# Autodesk Inventor assembly: Z assembly
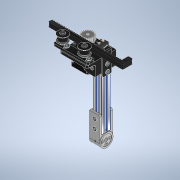
[picture p0: Inventor's stored thumbnail of the model, 180x180]
Saved by Autodesk Inventor 2022 (Build 260153000, 153)
## iProperties
Created: 2022-03-06
Part Number: Z assembly
Document SubType Name: Assembly
Designer: JK
Author: JK
## Documents named in this file (26)
- C:\Users\JK\Documents\Inventor\ScaraNema\SCARA-3DP\Parts\Forearm\Forearm assembly.iam
- C:\Users\JK\Documents\Inventor\ScaraNema\SCARA-3DP\Parts\Forearm\Z Motor support.ipt
- C:\Users\JK\Documents\Inventor\ScaraNema\SCARA-3DP\Parts\Forearm\Gear.ipt
- C:\Users\JK\Documents\Inventor\ScaraNema\SCARA-3DP\Parts\Forearm\Rack.ipt
- C:\Users\JK\Documents\Inventor\ScaraNema\SCARA-3DP\Parts\Common components\Motor.ipt
- C:\Users\JK\Documents\Inventor\ScaraNema\SCARA-3DP\Parts\V-Slot 20x20.ipt
- C:\Users\JK\Documents\Inventor\ScaraNema\SCARA-3DP\Parts\Forearm\Rack support.ipt
- C:\Users\JK\Documents\Inventor\ScaraNema\SCARA-3DP\Parts\Forearm\Roller.ipt
- C:\Users\JK\Documents\Inventor\ScaraNema\SCARA-3DP\Parts\Forearm\Z axis limit switch support.ipt
- C:\Users\JK\Documents\Inventor\ScaraNema\SCARA-3DP\Parts\Common components\V-Slot 20x20\V-Slot 20x20x150.ipt
- C:\Users\JK\Documents\Inventor\ScaraNema\SCARA-3DP\Parts\Arm\Soporte antebrazo.ipt
- C:\Users\JK\Documents\Inventor\ScaraNema\SCARA-3DP\Parts\Common components\Limit switch.ipt
- C:\Users\JK\Documents\Inventor\ScaraNema\SCARA-3DP\Parts\Fasteners\M2x10 socket bolt.ipt
- C:\Users\JK\Documents\Inventor\ScaraNema\SCARA-3DP\Parts\Fasteners\M2 Hex nut.ipt
- C:\Users\JK\Documents\Inventor\ScaraNema\SCARA-3DP\Parts\Fasteners\M3x10 set screw.ipt
- C:\Users\JK\Documents\Inventor\ScaraNema\SCARA-3DP\Parts\Fasteners\M5x15 Flat head bolt.ipt
- C:\Users\JK\Documents\Inventor\ScaraNema\SCARA-3DP\Parts\Fasteners\M5x10 Flat head bolt.ipt
- C:\Users\JK\Documents\Inventor\ScaraNema\SCARA-3DP\Parts\Fasteners\M5x8 Flat head bolt.ipt
- C:\Users\JK\Documents\Inventor\ScaraNema\SCARA-3DP\Parts\Fasteners\M3 Hex nut.ipt
- C:\Users\JK\Documents\Inventor\ScaraNema\SCARA-3DP\Parts\Fasteners\M5 Hex nut.ipt
- C:\Users\JK\Documents\Inventor\ScaraNema\SCARA-3DP\Parts\Common components\688-2RS.ipt
- C:\Users\JK\Documents\Inventor\ScaraNema\SCARA-3DP\Parts\Forearm\F623ZZ.ipt
- C:\Users\JK\Documents\Inventor\ScaraNema\SCARA-3DP\Parts\Fasteners\M3x25 socket solt.ipt
- C:\Users\JK\Documents\Inventor\ScaraNema\SCARA-3DP\Parts\Fasteners\M5 T-Nut Drop-in 20x20.ipt
- C:\Users\JK\Documents\Inventor\ScaraNema\SCARA-3DP\Parts\Forearm\Roller-bolt separator.ipt
- C:\Users\JK\Documents\Inventor\ScaraNema\SCARA-3DP\Parts\Fasteners\M3x6 socket bolt.ipt
## Components (61 placed, 24 different names)
1. Z Motor support:1 — Ángulo:2, Coincidencia:3, Ángulo:3, Coincidencia:4, Coincidencia:5, Nivelación:1, Coincidencia:6, Coincidencia:7, Nivelación:5, Coincidencia:32, Coincidencia:48, Coincidencia:49, Coincidencia:50, Coincidencia:51, Coincidencia:52, Ángulo:9, Coincidencia:56, Ángulo:19, Coincidencia:91, Coincidencia:92, Coincidencia:93, Coincidencia:94, Coincidencia:95, Coincidencia:96
2. Gear:1 — Coincidencia:1, Coincidencia:2, Coincidencia:3, Nivelación:2
3. Rack:1 — Ángulo:2, Nivelación:2, Nivelación:3, Tangente:1
4. Motor:1 — Coincidencia:1, Coincidencia:2, Ángulo:3, Coincidencia:4, Nivelación:3
5. V-Slot 20x20x150:1 — Coincidencia:5, Nivelación:1, Coincidencia:6, Coincidencia:16, Nivelación:8, Coincidencia:17, Coincidencia:18, Coincidencia:19, Coincidencia:29, Ángulo:12
6. Rack support:1 — Coincidencia:7, Nivelación:5, Coincidencia:39, Coincidencia:40, Ángulo:6, Coincidencia:41, Coincidencia:53, Coincidencia:61, Coincidencia:62, Coincidencia:63
7. Roller:1 — Nivelación:7, Tangente:1, Coincidencia:57, Coincidencia:60, Coincidencia:61, Nivelación:18, Coincidencia:64, Coincidencia:66
8. Roller:2 — Nivelación:7, Coincidencia:58, Coincidencia:59, Coincidencia:62, Nivelación:18, Coincidencia:65
9. Z axis limit switch support:1 — Coincidencia:16, Nivelación:8, Coincidencia:20, Coincidencia:21, Coincidencia:22, Ángulo:5, Coincidencia:28, Coincidencia:29, Coincidencia:46, Coincidencia:47, Coincidencia:89, Coincidencia:90
10. Soporte antebrazo:1 — Coincidencia:17, Coincidencia:18, Coincidencia:19, Coincidencia:33, Coincidencia:34, Coincidencia:35, Coincidencia:36, Coincidencia:37, Coincidencia:38, Coincidencia:42, Ángulo:8, Coincidencia:43, Coincidencia:44, Coincidencia:45, Ángulo:15, Coincidencia:83, Coincidencia:84, Coincidencia:85, Coincidencia:86, Coincidencia:87, Coincidencia:88
11. Limit switch:1 — Coincidencia:20, Coincidencia:21, Coincidencia:22, Coincidencia:23, Coincidencia:24, Coincidencia:25
12. M2x10 socket bolt:1 — Coincidencia:23, Nivelación:9, Coincidencia:26
13. M2x10 socket bolt:2 — Coincidencia:24, Nivelación:9, Coincidencia:25, Coincidencia:27
14. M2 Hex nut:1 — Coincidencia:27, Nivelación:10, Ángulo:4, Ángulo:5
15. M2 Hex nut:2 — Coincidencia:26, Nivelación:10, Ángulo:4, Coincidencia:28
16. M5x15 Flat head bolt:1 — Coincidencia:32, Coincidencia:73, Coincidencia:93
17. M5x10 Flat head bolt:1 — Coincidencia:33, Nivelación:12, Coincidencia:82, Coincidencia:86
18. M5x10 Flat head bolt:2 — Coincidencia:34, Nivelación:12, Coincidencia:81
19. M5x10 Flat head bolt:3 — Coincidencia:35, Nivelación:11, Coincidencia:77, Coincidencia:88
20. M5x10 Flat head bolt:4 — Coincidencia:36, Nivelación:11, Coincidencia:78
21. M5x8 Flat head bolt:1 — Coincidencia:37, Nivelación:13, Coincidencia:79, Coincidencia:87
22. M5x8 Flat head bolt:2 — Coincidencia:38, Nivelación:13, Coincidencia:80
23. M3 Hex nut:2 — Coincidencia:40, Nivelación:14, Ángulo:6, Ángulo:7, Coincidencia:41
24. M3 Hex nut:3 — Coincidencia:39, Nivelación:14, Ángulo:7
25. M5x8 Flat head bolt:3 — Coincidencia:47, Nivelación:15, Coincidencia:75, Coincidencia:90
26. M5x8 Flat head bolt:4 — Coincidencia:46, Nivelación:15, Coincidencia:74
27. M5x15 Flat head bolt:2 — Coincidencia:48, Coincidencia:76, Coincidencia:94
28. M5x15 Flat head bolt:3 — Coincidencia:49, Coincidencia:50
29. M5x10 Flat head bolt:5 — Coincidencia:52, Nivelación:16, Coincidencia:54
30. M5x10 Flat head bolt:6 — Coincidencia:51, Nivelación:16, Coincidencia:53, Coincidencia:55
31. M5 Hex nut:1 — Coincidencia:54, Nivelación:17, Ángulo:9, Ángulo:10
32. M5 Hex nut:2 — Coincidencia:55, Nivelación:17, Ángulo:10, Coincidencia:56
33. 688-2RS:1 — Coincidencia:57, Coincidencia:60, Coincidencia:63
34. 688-2RS:2 — Coincidencia:58, Coincidencia:59
35. F623ZZ:1 — Coincidencia:64, Nivelación:19, Coincidencia:66, Coincidencia:67, Coincidencia:69, Coincidencia:70
36. F623ZZ:2 — Coincidencia:65, Nivelación:19, Coincidencia:68
37. Roller-bolt separator:1 — Coincidencia:67, Coincidencia:69, Nivelación:20, Coincidencia:72
38. Roller-bolt separator:2 — Coincidencia:68, Nivelación:20, Coincidencia:71
39. M3x25 socket solt:1 — Coincidencia:71, Nivelación:21
40. M3x25 socket solt:2 — Coincidencia:70, Nivelación:21, Coincidencia:72
41. M5 T-Nut Drop-in 20x20:1 — Coincidencia:73, Coincidencia:91
42. M5 T-Nut Drop-in 20x20:2 — Coincidencia:74, Nivelación:22, Ángulo:18, Ángulo:19
43. M5 T-Nut Drop-in 20x20:3 — Coincidencia:75, Nivelación:22, Ángulo:18, Coincidencia:89
44. M5 T-Nut Drop-in 20x20:4 — Coincidencia:76, Coincidencia:92
45. M5 T-Nut Drop-in 20x20:5 — Coincidencia:77, Ángulo:13, Nivelación:25, Ángulo:14, Ángulo:17, Coincidencia:84
46. M5 T-Nut Drop-in 20x20:6 — Coincidencia:78, Ángulo:13, Nivelación:25, Ángulo:14, Ángulo:15
47. M5 T-Nut Drop-in 20x20:7 — Coincidencia:79, Nivelación:23, Ángulo:11, Coincidencia:85
48. M5 T-Nut Drop-in 20x20:8 — Coincidencia:80, Nivelación:23, Ángulo:11, Ángulo:12
49. M5 T-Nut Drop-in 20x20:9 — Coincidencia:82, Nivelación:24, Ángulo:16, Coincidencia:83
50. M5 T-Nut Drop-in 20x20:10 — Coincidencia:81, Nivelación:24, Ángulo:16, Ángulo:17
51. M3x6 socket bolt:1
52. M3x10 set screw:5 — Coincidencia:44, Coincidencia:45
53. M3 Hex nut:1 — Coincidencia:42, Ángulo:8, Coincidencia:43
54. M3x10 set screw:6
55. M3 Hex nut:4
56. M3x10 set screw:7
57. M3 Hex nut:5
58. M3x6 socket bolt:2 — Coincidencia:95, Coincidencia:96
59. M3x6 socket bolt:3
60. M3x6 socket bolt:4
61. M3x6 socket bolt:5
## Component patterns: (3 elements, first: M3x10 set screw:5 + M3 Hex nut:1), (4 elements, first: M3x6 socket bolt:2)
## Relationships (128: Mate 86, Flush 23, Angle 18, Tangent 1)
- Ángulo:2 [Angle] (180 deg): Z Motor support:1 ↔ Rack:1
- Coincidencia:1 [Mate]: Gear:1 ↔ Motor:1
- Coincidencia:2 [Mate] (2.5 mm): Gear:1 ↔ Motor:1
- Coincidencia:3 [Mate]: Z Motor support:1 ↔ Gear:1
- Ángulo:3 [Angle] (0 deg): Z Motor support:1 ↔ Motor:1
- Coincidencia:4 [Mate]: Z Motor support:1 ↔ Motor:1
- Coincidencia:5 [Mate]: Z Motor support:1 ↔ V-Slot 20x20x150:1
- Nivelación:1 [Flush]: Z Motor support:1 ↔ V-Slot 20x20x150:1
- Coincidencia:6 [Mate]: Z Motor support:1 ↔ V-Slot 20x20x150:1
- Nivelación:2 [Flush]: Gear:1 ↔ Rack:1
- Nivelación:3 [Flush] (-0.5 mm): Rack:1 ↔ Motor:1
- Coincidencia:7 [Mate]: Z Motor support:1 ↔ Rack support:1
- Nivelación:5 [Flush]: Z Motor support:1 ↔ Rack support:1
- Nivelación:7 [Flush]: Roller:1 ↔ Roller:2
- Coincidencia:16 [Mate]: V-Slot 20x20x150:1 ↔ Z axis limit switch support:1
- Nivelación:8 [Flush]: V-Slot 20x20x150:1 ↔ Z axis limit switch support:1
- Coincidencia:17 [Mate]: V-Slot 20x20x150:1 ↔ Soporte antebrazo:1
- Coincidencia:18 [Mate] (0.15 mm): V-Slot 20x20x150:1 ↔ Soporte antebrazo:1
- Coincidencia:19 [Mate]: V-Slot 20x20x150:1 ↔ Soporte antebrazo:1
- Coincidencia:20 [Mate]: Z axis limit switch support:1 ↔ Limit switch:1
- Coincidencia:21 [Mate]: Z axis limit switch support:1 ↔ Limit switch:1
- Coincidencia:22 [Mate]: Z axis limit switch support:1 ↔ Limit switch:1
- Coincidencia:23 [Mate]: Limit switch:1 ↔ M2x10 socket bolt:1
- Coincidencia:24 [Mate]: Limit switch:1 ↔ M2x10 socket bolt:2
- Nivelación:9 [Flush]: M2x10 socket bolt:1 ↔ M2x10 socket bolt:2
- Coincidencia:25 [Mate]: Limit switch:1 ↔ M2x10 socket bolt:2
- Coincidencia:26 [Mate]: M2x10 socket bolt:1 ↔ M2 Hex nut:2
- Coincidencia:27 [Mate]: M2x10 socket bolt:2 ↔ M2 Hex nut:1
- Nivelación:10 [Flush]: M2 Hex nut:1 ↔ M2 Hex nut:2
- Ángulo:4 [Angle] (0 deg): M2 Hex nut:1 ↔ M2 Hex nut:2
- Ángulo:5 [Angle] (0 deg): Z axis limit switch support:1 ↔ M2 Hex nut:1
- Coincidencia:28 [Mate]: Z axis limit switch support:1 ↔ M2 Hex nut:2
- Coincidencia:29 [Mate] (10 mm): V-Slot 20x20x150:1 ↔ Z axis limit switch support:1
- Coincidencia:32 [Mate]: Z Motor support:1 ↔ M5x15 Flat head bolt:1
- Coincidencia:33 [Mate]: Soporte antebrazo:1 ↔ M5x10 Flat head bolt:1
- Coincidencia:34 [Mate]: Soporte antebrazo:1 ↔ M5x10 Flat head bolt:2
- Coincidencia:35 [Mate]: Soporte antebrazo:1 ↔ M5x10 Flat head bolt:3
- Coincidencia:36 [Mate]: Soporte antebrazo:1 ↔ M5x10 Flat head bolt:4
- Nivelación:11 [Flush]: M5x10 Flat head bolt:3 ↔ M5x10 Flat head bolt:4
- Nivelación:12 [Flush]: M5x10 Flat head bolt:1 ↔ M5x10 Flat head bolt:2
- Coincidencia:37 [Mate]: Soporte antebrazo:1 ↔ M5x8 Flat head bolt:1
- Coincidencia:38 [Mate]: Soporte antebrazo:1 ↔ M5x8 Flat head bolt:2
- Nivelación:13 [Flush]: M5x8 Flat head bolt:1 ↔ M5x8 Flat head bolt:2
- Coincidencia:39 [Mate]: Rack support:1 ↔ M3 Hex nut:3
- Coincidencia:40 [Mate]: Rack support:1 ↔ M3 Hex nut:2
- Nivelación:14 [Flush]: M3 Hex nut:2 ↔ M3 Hex nut:3
- Ángulo:6 [Angle] (0 deg): Rack support:1 ↔ M3 Hex nut:2
- Ángulo:7 [Angle] (0 deg): M3 Hex nut:2 ↔ M3 Hex nut:3
- Coincidencia:41 [Mate]: Rack support:1 ↔ M3 Hex nut:2
- Coincidencia:42 [Mate]: Soporte antebrazo:1 ↔ M3 Hex nut:1
- Ángulo:8 [Angle] (0 deg): Soporte antebrazo:1 ↔ M3 Hex nut:1
- Coincidencia:43 [Mate]: Soporte antebrazo:1 ↔ M3 Hex nut:1
- Coincidencia:44 [Mate]: Soporte antebrazo:1 ↔ M3x10 set screw:5
- Coincidencia:45 [Mate] (-5 mm): Soporte antebrazo:1 ↔ M3x10 set screw:5
- Coincidencia:46 [Mate]: Z axis limit switch support:1 ↔ M5x8 Flat head bolt:4
- Coincidencia:47 [Mate]: Z axis limit switch support:1 ↔ M5x8 Flat head bolt:3
- Nivelación:15 [Flush]: M5x8 Flat head bolt:3 ↔ M5x8 Flat head bolt:4
- Coincidencia:48 [Mate]: Z Motor support:1 ↔ M5x15 Flat head bolt:2
- Coincidencia:49 [Mate]: Z Motor support:1 ↔ M5x15 Flat head bolt:3
- Coincidencia:50 [Mate]: Z Motor support:1 ↔ M5x15 Flat head bolt:3
- Tangente:1: Rack:1 ↔ Roller:1
- Coincidencia:51 [Mate]: Z Motor support:1 ↔ M5x10 Flat head bolt:6
- Coincidencia:52 [Mate]: Z Motor support:1 ↔ M5x10 Flat head bolt:5
- Nivelación:16 [Flush]: M5x10 Flat head bolt:5 ↔ M5x10 Flat head bolt:6
- Coincidencia:53 [Mate]: Rack support:1 ↔ M5x10 Flat head bolt:6
- Coincidencia:54 [Mate]: M5x10 Flat head bolt:5 ↔ M5 Hex nut:1
- Coincidencia:55 [Mate]: M5x10 Flat head bolt:6 ↔ M5 Hex nut:2
- Nivelación:17 [Flush]: M5 Hex nut:1 ↔ M5 Hex nut:2
- Ángulo:9 [Angle] (0 deg): Z Motor support:1 ↔ M5 Hex nut:1
- Ángulo:10 [Angle] (0 deg): M5 Hex nut:1 ↔ M5 Hex nut:2
- Coincidencia:56 [Mate]: Z Motor support:1 ↔ M5 Hex nut:2
- Coincidencia:57 [Mate]: Roller:1 ↔ 688-2RS:1
- Coincidencia:58 [Mate]: Roller:2 ↔ 688-2RS:2
- Coincidencia:59 [Mate]: Roller:2 ↔ 688-2RS:2
- Coincidencia:60 [Mate]: Roller:1 ↔ 688-2RS:1
- Coincidencia:61 [Mate]: Rack support:1 ↔ Roller:1
- Coincidencia:62 [Mate]: Rack support:1 ↔ Roller:2
- Nivelación:18 [Flush]: Roller:1 ↔ Roller:2
- Coincidencia:63 [Mate]: Rack support:1 ↔ 688-2RS:1
- Coincidencia:64 [Mate]: Roller:1 ↔ F623ZZ:1
- Coincidencia:65 [Mate]: Roller:2 ↔ F623ZZ:2
- Nivelación:19 [Flush]: F623ZZ:1 ↔ F623ZZ:2
- Coincidencia:66 [Mate]: Roller:1 ↔ F623ZZ:1
- Coincidencia:67 [Mate]: F623ZZ:1 ↔ Roller-bolt separator:1
- Coincidencia:68 [Mate]: F623ZZ:2 ↔ Roller-bolt separator:2
- Coincidencia:69 [Mate]: F623ZZ:1 ↔ Roller-bolt separator:1
- Nivelación:20 [Flush]: Roller-bolt separator:1 ↔ Roller-bolt separator:2
- Coincidencia:70 [Mate]: F623ZZ:1 ↔ M3x25 socket solt:2
- Coincidencia:71 [Mate]: Roller-bolt separator:2 ↔ M3x25 socket solt:1
- Nivelación:21 [Flush]: M3x25 socket solt:1 ↔ M3x25 socket solt:2
- Coincidencia:72 [Mate]: Roller-bolt separator:1 ↔ M3x25 socket solt:2
- Coincidencia:73 [Mate]: M5x15 Flat head bolt:1 ↔ M5 T-Nut Drop-in 20x20:1
- Coincidencia:74 [Mate]: M5x8 Flat head bolt:4 ↔ M5 T-Nut Drop-in 20x20:2
- Coincidencia:75 [Mate]: M5x8 Flat head bolt:3 ↔ M5 T-Nut Drop-in 20x20:3
- Coincidencia:76 [Mate]: M5x15 Flat head bolt:2 ↔ M5 T-Nut Drop-in 20x20:4
- Nivelación:22 [Flush]: M5 T-Nut Drop-in 20x20:2 ↔ M5 T-Nut Drop-in 20x20:3
- Coincidencia:77 [Mate]: M5x10 Flat head bolt:3 ↔ M5 T-Nut Drop-in 20x20:5
- Coincidencia:78 [Mate]: M5x10 Flat head bolt:4 ↔ M5 T-Nut Drop-in 20x20:6
- Coincidencia:79 [Mate]: M5x8 Flat head bolt:1 ↔ M5 T-Nut Drop-in 20x20:7
- Coincidencia:80 [Mate]: M5x8 Flat head bolt:2 ↔ M5 T-Nut Drop-in 20x20:8
- Coincidencia:81 [Mate]: M5x10 Flat head bolt:2 ↔ M5 T-Nut Drop-in 20x20:10
- Coincidencia:82 [Mate]: M5x10 Flat head bolt:1 ↔ M5 T-Nut Drop-in 20x20:9
- Nivelación:23 [Flush]: M5 T-Nut Drop-in 20x20:7 ↔ M5 T-Nut Drop-in 20x20:8
- Nivelación:24 [Flush]: M5 T-Nut Drop-in 20x20:9 ↔ M5 T-Nut Drop-in 20x20:10
- Ángulo:11 [Angle] (0 deg): M5 T-Nut Drop-in 20x20:7 ↔ M5 T-Nut Drop-in 20x20:8
- Ángulo:12 [Angle] (90 deg): V-Slot 20x20x150:1 ↔ M5 T-Nut Drop-in 20x20:8
- Ángulo:13 [Angle] (0 deg): M5 T-Nut Drop-in 20x20:5 ↔ M5 T-Nut Drop-in 20x20:6
- Nivelación:25 [Flush]: M5 T-Nut Drop-in 20x20:5 ↔ M5 T-Nut Drop-in 20x20:6
- Ángulo:14 [Angle] (0 deg): M5 T-Nut Drop-in 20x20:5 ↔ M5 T-Nut Drop-in 20x20:6
- Ángulo:15 [Angle] (0 deg): Soporte antebrazo:1 ↔ M5 T-Nut Drop-in 20x20:6
- Ángulo:16 [Angle] (0 deg): M5 T-Nut Drop-in 20x20:9 ↔ M5 T-Nut Drop-in 20x20:10
- Ángulo:17 [Angle] (0 deg): M5 T-Nut Drop-in 20x20:5 ↔ M5 T-Nut Drop-in 20x20:10
- Coincidencia:83 [Mate] (0.6 mm): Soporte antebrazo:1 ↔ M5 T-Nut Drop-in 20x20:9
- Coincidencia:84 [Mate] (0.6 mm): Soporte antebrazo:1 ↔ M5 T-Nut Drop-in 20x20:5
- Coincidencia:85 [Mate] (0.6 mm): Soporte antebrazo:1 ↔ M5 T-Nut Drop-in 20x20:7
- Coincidencia:86 [Mate]: Soporte antebrazo:1 ↔ M5x10 Flat head bolt:1
- Coincidencia:87 [Mate]: Soporte antebrazo:1 ↔ M5x8 Flat head bolt:1
- Coincidencia:88 [Mate]: Soporte antebrazo:1 ↔ M5x10 Flat head bolt:3
- Ángulo:18 [Angle] (0 deg): M5 T-Nut Drop-in 20x20:2 ↔ M5 T-Nut Drop-in 20x20:3
- Ángulo:19 [Angle] (0 deg): Z Motor support:1 ↔ M5 T-Nut Drop-in 20x20:2
- Coincidencia:89 [Mate] (0.6 mm): Z axis limit switch support:1 ↔ M5 T-Nut Drop-in 20x20:3
- Coincidencia:90 [Mate]: Z axis limit switch support:1 ↔ M5x8 Flat head bolt:3
- Coincidencia:91 [Mate] (0.6 mm): Z Motor support:1 ↔ M5 T-Nut Drop-in 20x20:1
- Coincidencia:92 [Mate] (0.6 mm): Z Motor support:1 ↔ M5 T-Nut Drop-in 20x20:4
- Coincidencia:93 [Mate]: Z Motor support:1 ↔ M5x15 Flat head bolt:1
- Coincidencia:94 [Mate]: Z Motor support:1 ↔ M5x15 Flat head bolt:2
- Coincidencia:95 [Mate]: Z Motor support:1 ↔ M3x6 socket bolt:2
- Coincidencia:96 [Mate]: Z Motor support:1 ↔ M3x6 socket bolt:2
